# Autodesk Inventor assembly: 305-07
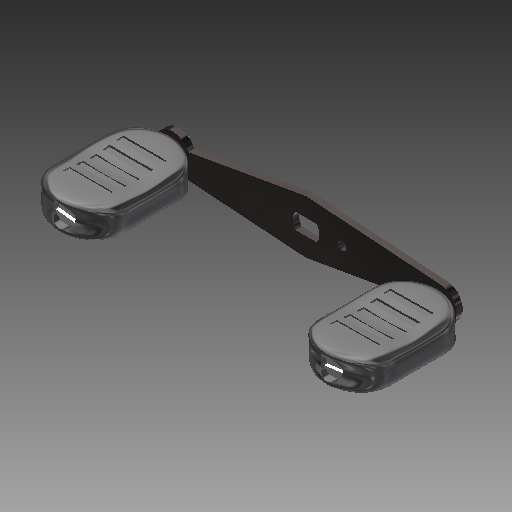
[picture p0: Inventor's stored thumbnail of the model, 512x512]
Saved by Autodesk Inventor 2019 (Build 230136000, 136)
## iProperties
Company: Autodesk Inc.
Created: 2012-01-25
Part Number: 305-07
Document SubType Name: Assembly
Designer: Autodesk Inc.
Mass: 22.5168 g
Surface Area: 86.6693 cm^2
Volume: 12.5205 cm^3
Density: 1.79839 g/cm^3
Author: Inventor
## Documents named in this file (4)
- C:\TEMP\Fishing Rod\Workspaces\Winding Handle.iam
- C:\TEMP\Fishing Rod\Workspaces\Winding Handle.ipt
- C:\TEMP\Fishing Rod\Workspaces\Grip Spindle.ipt
- C:\TEMP\Fishing Rod\Workspaces\Grip.ipt
## Components (5 placed, 3 different names)
1. Winding Handle:1 — Insert:1, Insert:2
2. Grip Spindle:1 — Insert:1, Insert:6
3. Grip Spindle:2 — Insert:2, Insert:5
4. Grip:1 — Insert:6
5. Grip:2 — Insert:5
## Relationships (4: Insert 4)
- Insert:1: Winding Handle:1 ↔ Grip Spindle:1
- Insert:2: Winding Handle:1 ↔ Grip Spindle:2
- Insert:5: Grip Spindle:2 ↔ Grip:2
- Insert:6: Grip Spindle:1 ↔ Grip:1
